# Autodesk Inventor assembly: DriveSystem
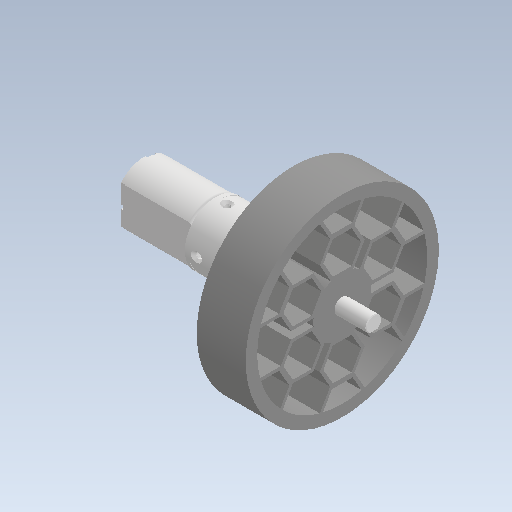
[picture p0: Inventor's stored thumbnail of the model, 512x512]
Saved by Autodesk Inventor 2020 (Build 240168000, 168)
## iProperties
Created: 2024-02-19
Part Number: DriveSystem
Document SubType Name: Assembly
Designer: smz3rm
Author: smz3rm
## Documents named in this file (3)
- C:\Users\smz3rm\OneDrive - BP\Documents\Battlebots\VerticalSpinner\DriveSystem.iam
- C:\Users\smz3rm\OneDrive - BP\Documents\Battlebots\VerticalSpinner\VertWheelV1.ipt
- C:\Users\smz3rm\OneDrive - BP\Documents\Battlebots\VerticalSpinner\RepeatDriveBrushedMk2 - 4mm.iam
## Components (2 placed, 2 different names)
1. VertWheelV1:1 — Mate:1, Mate:2
2. RepeatDriveBrushedMk2 - 4mm:1 [sub-assembly] — Mate:1, Mate:2
## Relationships (2: Mate 2)
- Mate:1: VertWheelV1:1 ↔ RepeatDriveBrushedMk2 - 4mm:1
- Mate:2 (0.5 mm): VertWheelV1:1 ↔ RepeatDriveBrushedMk2 - 4mm:1
